# Autodesk Inventor assembly: plate+resistors
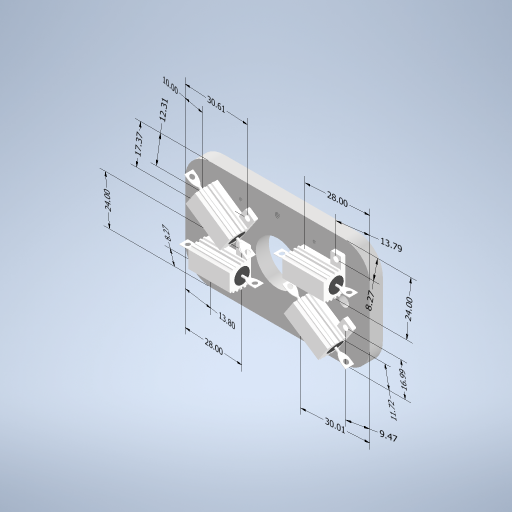
[picture p0: Inventor's stored thumbnail of the model, 512x512]
Saved by Autodesk Inventor 2024 (Build 280153000, 153)
## iProperties
Created: 2023-09-14
Part Number: plate+resistors
Document SubType Name: Assembly
Designer: raad
Author: raad
## Documents named in this file (3)
- C:\Users\Fujitsu\Raad\BaTag\camera\plate+resistors.iam
- C:\Users\Fujitsu\Raad\BaTag\camera\new-adapter-plate.ipt
- C:\Users\Fujitsu\Raad\BaTag\camera\RH-NH010\RH-NH010.ipt
## Components (5 placed, 2 different names)
1. new-adapter-plate:1 — Mate:1, Mate:2, Mate:3, Mate:4
2. RH-NH010:1 — Mate:1
3. RH-NH010:2 — Mate:2
4. RH-NH010:3 — Mate:3
5. RH-NH010:4 — Mate:4
## Relationships (4: Mate 4)
- Mate:1: new-adapter-plate:1 ↔ RH-NH010:1
- Mate:2: new-adapter-plate:1 ↔ RH-NH010:2
- Mate:3: new-adapter-plate:1 ↔ RH-NH010:3
- Mate:4: new-adapter-plate:1 ↔ RH-NH010:4
